# Autodesk Inventor assembly: Body
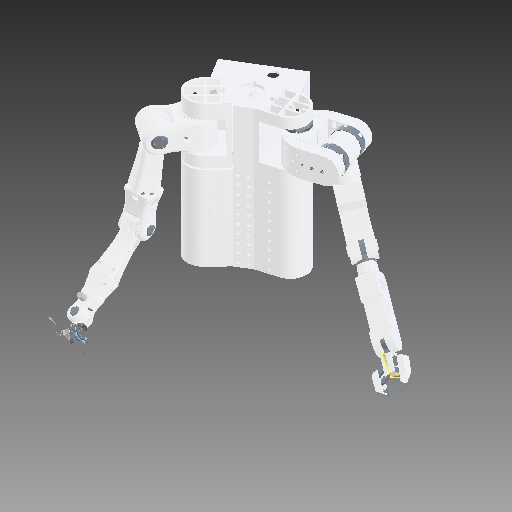
[picture p0: Inventor's stored thumbnail of the model, 512x512]
Saved by Autodesk Inventor 2017 SP1 (Build 210196100, 196)
## iProperties
Created: 2017-03-13
Part Number: Body
Document SubType Name: Assembly
Designer: zallen
Author: zallen
## Documents named in this file (4)
- C:\Users\Zach\Documents\GitHub\tr1\src\Body\Body.iam
- C:\Users\Zach\Documents\GitHub\tr1\src\Body\Arm Assembly\ArmAssembly.iam
- C:\Users\Zach\Documents\GitHub\tr1\src\Body\Chest Assembly\Chest Assembly.iam
- C:\Users\Zach\Documents\GitHub\tr1\src\Body\Arm 2.0 Assembly\Arm 2.0 Assembly.iam
## Components (3 placed, 3 different names)
1. ArmAssembly:1 [sub-assembly] — Mate:1, Mate:2
2. Chest Assembly:1 [sub-assembly] — Mate:1, Mate:2, Mate:3, Mate:4
3. Arm 2.0 Assembly:1 [sub-assembly] — Mate:3, Mate:4
## Relationships (4: Mate 4)
- Mate:1: ArmAssembly:1 ↔ Chest Assembly:1
- Mate:2: ArmAssembly:1 ↔ Chest Assembly:1
- Mate:3: Chest Assembly:1 ↔ Arm 2.0 Assembly:1
- Mate:4: Chest Assembly:1 ↔ Arm 2.0 Assembly:1
